# Autodesk Inventor assembly: Multipass-1
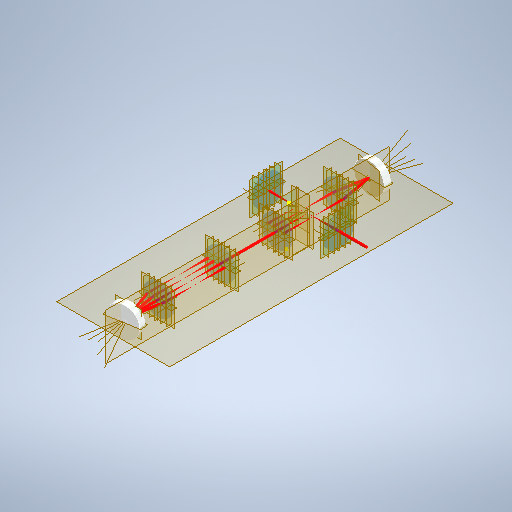
[picture p0: Inventor's stored thumbnail of the model, 512x512]
Saved by Autodesk Inventor 2025 (Build 290162010, 162A)
## iProperties
Created: 2024-08-12
Part Number: Multipass-1
Document SubType Name: Assembly
Designer: User
Author: User
## Documents named in this file (10)
- C:\Users\User\Desktop\Hari_Laptop_Contents\KerlinLab\KTN\Multipass\MechanicalDrawing\Multipass-1.iam
- C:\Users\User\Desktop\Hari_Laptop_Contents\KerlinLab\KTN\Multipass\MechanicalDrawing\LA1608-AB-Solidworks\LA1608-AB-Solidworks.ipt
- C:\Users\User\Desktop\Hari_Laptop_Contents\KerlinLab\KTN\Multipass\MechanicalDrawing\BB1-E02-Solidworks.ipt
- C:\Users\User\Desktop\Hari_Laptop_Contents\KerlinLab\KTN\Multipass\MechanicalDrawing\ExitMirror.ipt
- C:\Users\User\Desktop\Hari_Laptop_Contents\KerlinLab\KTN\Multipass\MechanicalDrawing\EntryMirror.ipt
- C:\Users\User\Desktop\Hari_Laptop_Contents\KerlinLab\KTN\Multipass\MechanicalDrawing\LaserBeamEntry1.ipt
- C:\Users\User\Desktop\Hari_Laptop_Contents\KerlinLab\KTN\Multipass\MechanicalDrawing\LaserBeamEntry2.ipt
- C:\Users\User\Desktop\Hari_Laptop_Contents\KerlinLab\KTN\Multipass\MechanicalDrawing\LaserBeam3.ipt
- C:\Users\User\Desktop\Hari_Laptop_Contents\KerlinLab\KTN\Multipass\MechanicalDrawing\LaserBeam4.ipt
- C:\Users\User\Desktop\Hari_Laptop_Contents\KerlinLab\KTN\Multipass\MechanicalDrawing\LaserBeam5.ipt
## Components (34 placed, 9 different names)
1. LA1608-AB-Solidworks:1 — Mate:1, Mate:4, Mate:9, Mate:10, Mate:11, Mate:12, Mate:13, Mate:45, Mate:54, Mate:60, Mate:87, Mate:88, Mate:89, Mate:90
2. LA1608-AB-Solidworks:2 — Mate:1, Mate:2, Mate:3, Mate:6, Mate:32, Mate:34, Mate:47, Mate:50, Mate:56, Mate:61, Mate:62, Mate:63, Mate:64, Mate:65, Mate:66, Mate:77, Mate:78
3. LA1608-AB-Solidworks:3 — Mate:2, Mate:5, Mate:6, Mate:30, Mate:47, Mate:48, Mate:51, Mate:68, Mate:69, Mate:71, Mate:72, Mate:73, Mate:74, Mate:75, Mate:76
4. LA1608-AB-Solidworks:4 — Mate:10, Mate:11, Mate:16, Mate:18, Mate:91, Mate:92, Mate:93
5. LA1608-AB-Solidworks:5 — Mate:3, Mate:4, Mate:5, Mate:15, Mate:17, Mate:24, Mate:25, Mate:31, Mate:48, Mate:52, Mate:81, Mate:82, Mate:83, Mate:84, Mate:85, Mate:86
6. LA1608-AB-Solidworks:6 — Mate:12, Mate:13, Angle:1, Mate:21, Mate:22, Mate:53, Mate:58, Mate:59
7. BB1-E02-Solidworks:1 — Mate:9, Mate:40, Mate:41, Mate:42, Mate:45, Mate:55
8. BB1-E02-Solidworks:2 — Mate:32, Mate:33, Mate:34, Mate:36, Mate:37, Mate:38, Mate:39, Mate:43, Mate:46, Mate:49
9. ExitMirror:1 — Mate:18, Mate:20, Mate:60
10. EntryMirror:1 — Angle:1, Mate:15, Mate:16, Mate:17, Mate:20
11. LaserBeamEntry1:1 — Mate:21, Mate:23, Mate:58
12. LaserBeamEntry2:1 — Mate:22, Mate:23, Mate:59
13. LaserBeamEntry2:2 — Mate:24, Mate:25
14. LaserBeam3:1 — Mate:30, Mate:31
15. LaserBeam4:1 — Mate:33, Mate:57
16. LaserBeam5:1 — Mate:36, Mate:37, Mate:57
17. LaserBeam5:2 — Mate:39, Mate:43
18. LaserBeam5:3 — Mate:41, Mate:42, Mate:44
19. LaserBeam5:4 — Mate:40, Mate:44
20. LaserBeam5:5 — Mate:38, Mate:46
21. LaserBeamEntry2:3 — Mate:63, Mate:64
22. LaserBeamEntry2:4 — Mate:73, Mate:74
23. LaserBeamEntry2:5 — Mate:68, Mate:72
24. LaserBeamEntry2:6 — Mate:69, Mate:71
25. LaserBeamEntry2:7 — Mate:77, Mate:78
26. LaserBeamEntry2:8 — Mate:81, Mate:86
27. LaserBeamEntry2:9 — Mate:61, Mate:62
28. LaserBeamEntry2:10 — Mate:65, Mate:66
29. LaserBeamEntry2:11 — Mate:75, Mate:76
30. LaserBeamEntry2:12 — Mate:83, Mate:84
31. LaserBeamEntry2:13 — Mate:82, Mate:85
32. LaserBeamEntry2:14 — Mate:87, Mate:90
33. LaserBeamEntry2:15 — Mate:91, Mate:92
34. LaserBeamEntry2:16 — Mate:88, Mate:89
## Relationships (81: Mate 80, Angle 1)
- Mate:1: LA1608-AB-Solidworks:1 ↔ LA1608-AB-Solidworks:2
- Mate:2: LA1608-AB-Solidworks:2 ↔ LA1608-AB-Solidworks:3
- Mate:3: LA1608-AB-Solidworks:2 ↔ LA1608-AB-Solidworks:5
- Mate:4 (50 mm): LA1608-AB-Solidworks:1 ↔ LA1608-AB-Solidworks:5
- Mate:5 (-50 mm): LA1608-AB-Solidworks:3 ↔ LA1608-AB-Solidworks:5
- Mate:6 (50 mm): LA1608-AB-Solidworks:2 ↔ LA1608-AB-Solidworks:3
- Mate:9: LA1608-AB-Solidworks:1 ↔ BB1-E02-Solidworks:1
- Mate:10 (-35 mm): LA1608-AB-Solidworks:1 ↔ LA1608-AB-Solidworks:4
- Mate:11 (25 mm): LA1608-AB-Solidworks:1 ↔ LA1608-AB-Solidworks:4
- Mate:12 (25 mm): LA1608-AB-Solidworks:1 ↔ LA1608-AB-Solidworks:6
- Mate:13 (25 mm): LA1608-AB-Solidworks:1 ↔ LA1608-AB-Solidworks:6
- Angle:1 (135 deg): LA1608-AB-Solidworks:6 ↔ EntryMirror:1
- Mate:15 (-1.5 mm): LA1608-AB-Solidworks:5 ↔ EntryMirror:1
- Mate:16: LA1608-AB-Solidworks:4 ↔ EntryMirror:1
- Mate:17: LA1608-AB-Solidworks:5 ↔ EntryMirror:1
- Mate:18: LA1608-AB-Solidworks:4 ↔ ExitMirror:1
- Mate:20: ExitMirror:1 ↔ EntryMirror:1
- Mate:21: LA1608-AB-Solidworks:6 ↔ LaserBeamEntry1:1
- Mate:22: LA1608-AB-Solidworks:6 ↔ LaserBeamEntry2:1
- Mate:23: LaserBeamEntry1:1 ↔ LaserBeamEntry2:1
- Mate:24: LA1608-AB-Solidworks:5 ↔ LaserBeamEntry2:2
- Mate:25: LA1608-AB-Solidworks:5 ↔ LaserBeamEntry2:2
- Mate:30: LA1608-AB-Solidworks:3 ↔ LaserBeam3:1
- Mate:31: LA1608-AB-Solidworks:5 ↔ LaserBeam3:1
- Mate:32: LA1608-AB-Solidworks:2 ↔ BB1-E02-Solidworks:2
- Mate:33: BB1-E02-Solidworks:2 ↔ LaserBeam4:1
- Mate:34 (25 mm): LA1608-AB-Solidworks:2 ↔ BB1-E02-Solidworks:2
- Mate:36: BB1-E02-Solidworks:2 ↔ LaserBeam5:1
- Mate:37: BB1-E02-Solidworks:2 ↔ LaserBeam5:1
- Mate:38: BB1-E02-Solidworks:2 ↔ LaserBeam5:5
- Mate:39: BB1-E02-Solidworks:2 ↔ LaserBeam5:2
- Mate:40: BB1-E02-Solidworks:1 ↔ LaserBeam5:4
- Mate:41: BB1-E02-Solidworks:1 ↔ LaserBeam5:3
- Mate:42: BB1-E02-Solidworks:1 ↔ LaserBeam5:3
- Mate:43: BB1-E02-Solidworks:2 ↔ LaserBeam5:2
- Mate:44: LaserBeam5:3 ↔ LaserBeam5:4
- Mate:45 (25 mm): LA1608-AB-Solidworks:1 ↔ BB1-E02-Solidworks:1
- Mate:46: BB1-E02-Solidworks:2 ↔ LaserBeam5:5
- Mate:47: LA1608-AB-Solidworks:2 ↔ LA1608-AB-Solidworks:3
- Mate:48: LA1608-AB-Solidworks:3 ↔ LA1608-AB-Solidworks:5
- Mate:49: BB1-E02-Solidworks:2
- Mate:50: LA1608-AB-Solidworks:2
- Mate:51: LA1608-AB-Solidworks:3
- Mate:52: LA1608-AB-Solidworks:5
- Mate:53: LA1608-AB-Solidworks:6
- Mate:54: LA1608-AB-Solidworks:1
- Mate:55: BB1-E02-Solidworks:1
- Mate:56: LA1608-AB-Solidworks:2
- Mate:57: LaserBeam4:1 ↔ LaserBeam5:1
- Mate:58: LA1608-AB-Solidworks:6 ↔ LaserBeamEntry1:1
- Mate:59: LA1608-AB-Solidworks:6 ↔ LaserBeamEntry2:1
- Mate:60: LA1608-AB-Solidworks:1 ↔ ExitMirror:1
- Mate:61: LA1608-AB-Solidworks:2 ↔ LaserBeamEntry2:9
- Mate:62: LA1608-AB-Solidworks:2 ↔ LaserBeamEntry2:9
- Mate:63: LA1608-AB-Solidworks:2 ↔ LaserBeamEntry2:3
- Mate:64: LA1608-AB-Solidworks:2 ↔ LaserBeamEntry2:3
- Mate:65: LA1608-AB-Solidworks:2 ↔ LaserBeamEntry2:10
- Mate:66: LA1608-AB-Solidworks:2 ↔ LaserBeamEntry2:10
- Mate:68: LA1608-AB-Solidworks:3 ↔ LaserBeamEntry2:5
- Mate:69: LA1608-AB-Solidworks:3 ↔ LaserBeamEntry2:6
- Mate:71: LA1608-AB-Solidworks:3 ↔ LaserBeamEntry2:6
- Mate:72: LA1608-AB-Solidworks:3 ↔ LaserBeamEntry2:5
- Mate:73: LA1608-AB-Solidworks:3 ↔ LaserBeamEntry2:4
- Mate:74: LA1608-AB-Solidworks:3 ↔ LaserBeamEntry2:4
- Mate:75: LA1608-AB-Solidworks:3 ↔ LaserBeamEntry2:11
- Mate:76: LA1608-AB-Solidworks:3 ↔ LaserBeamEntry2:11
- Mate:77: LA1608-AB-Solidworks:2 ↔ LaserBeamEntry2:7
- Mate:78: LA1608-AB-Solidworks:2 ↔ LaserBeamEntry2:7
- Mate:81: LA1608-AB-Solidworks:5 ↔ LaserBeamEntry2:8
- Mate:82: LA1608-AB-Solidworks:5 ↔ LaserBeamEntry2:13
- Mate:83: LA1608-AB-Solidworks:5 ↔ LaserBeamEntry2:12
- Mate:84: LA1608-AB-Solidworks:5 ↔ LaserBeamEntry2:12
- Mate:85: LA1608-AB-Solidworks:5 ↔ LaserBeamEntry2:13
- Mate:86: LA1608-AB-Solidworks:5 ↔ LaserBeamEntry2:8
- Mate:87: LA1608-AB-Solidworks:1 ↔ LaserBeamEntry2:14
- Mate:88: LA1608-AB-Solidworks:1 ↔ LaserBeamEntry2:16
- Mate:89: LA1608-AB-Solidworks:1 ↔ LaserBeamEntry2:16
- Mate:90: LA1608-AB-Solidworks:1 ↔ LaserBeamEntry2:14
- Mate:91: LA1608-AB-Solidworks:4 ↔ LaserBeamEntry2:15
- Mate:92: LA1608-AB-Solidworks:4 ↔ LaserBeamEntry2:15
- Mate:93: LA1608-AB-Solidworks:4
